# Autodesk Inventor assembly: Automoblox Car assembly
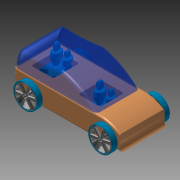
[picture p0: Inventor's stored thumbnail of the model, 180x180]
Saved by Autodesk Inventor 2015 (Build 190159000, 159)
## iProperties
Created: 2014-10-30
Part Number: Automoblox Car assembly
Document SubType Name: Assembly
Designer: cearhart275
Author: cearhart275
## Documents named in this file (14)
- H:\IED II\Automoblox Car assembly.iam
- H:\IED II\Body.ipt
- H:\IED II\Connector Piece.ipt
- H:\IED II\Front.ipt
- H:\IED II\Socket(ellipse Insert).ipt
- H:\IED II\Sockets(Rectangular insert).ipt
- H:\IED II\Tail.ipt
- H:\IED II\Passenger Base.ipt
- H:\IED II\Female Body.ipt
- H:\IED II\Male Figure.ipt
- H:\IED II\Windshield.ipt
- H:\IED II\Axle.ipt
- H:\IED II\Wheel.ipt
- H:\IED II\tire.ipt
## Components (28 placed, 13 different names)
1. Body:1 — Flush:1, Flush:2, Mate:1, Flush:3, Mate:2, Mate:3, Mate:4, Flush:4, Mate:12, Flush:8, Flush:9, Flush:10, Flush:11, Mate:16, Mate:17, Mate:18, Mate:22, Flush:13, Flush:14, Mate:23, Mate:29, Mate:35, Flush:18
2. Socket(ellipse Insert):1 — Flush:1, Flush:2, Mate:1, Flush:3, Mate:2, Mate:5, Mate:6, Mate:19
3. Sockets(Rectangular insert):1 — Mate:3, Mate:4, Flush:4, Mate:7
4. Connector Piece:1 — Mate:5, Mate:6, Mate:19
5. Connector Piece:2 — Mate:7
6. Tail:1 — Mate:8, Mate:9, Mate:10, Flush:5, Flush:6, Flush:7, Mate:11, Mate:12, Flush:8, Flush:9, Flush:10, Flush:11, Mate:13, Mate:14, Mate:15, Mate:26, Mate:32, Mate:36, Insert:3, Insert:4
7. Socket(ellipse Insert):2 — Mate:8, Mate:9, Mate:10, Flush:5, Flush:6, Flush:7, Mate:11
8. Passenger Base:1 — Mate:13, Mate:14, Mate:15, Mate:27, Mate:28, Mate:33, Mate:34, Flush:17
9. Passenger Base:2 — Mate:16, Mate:17, Mate:18, Mate:24, Mate:25, Mate:30, Mate:31, Flush:15, Flush:16
10. Front:1 — Mate:20, Mate:21, Flush:12, Mate:22, Flush:13, Flush:14, Insert:1, Mate:37, Insert:2
11. Sockets(Rectangular insert):2 — Mate:20, Mate:21, Flush:12
12. Male Figure:1 — Mate:23, Mate:24, Mate:25, Flush:16
13. Male Figure:2 — Mate:26, Mate:27, Mate:28
14. Female Body:1 — Mate:29, Mate:30, Mate:31, Flush:15
15. Female Body:2 — Mate:32, Mate:33, Mate:34, Flush:17
16. Windshield:1 — Mate:35, Flush:18, Mate:36
17. Axle:1 — Insert:1, Mate:37, Insert:5
18. Axle:2 — Insert:2, Insert:7
19. Axle:3 — Insert:3, Insert:6
20. Axle:4 — Insert:4, Insert:8
21. Wheel:1 — Mate:38, Flush:19, Insert:5
22. tire:1 — Mate:38, Flush:19
23. tire:2 — Mate:39, Flush:20
24. tire:3 — Mate:41, Flush:22
25. tire:4 — Mate:40, Flush:21
26. Wheel:2 — Mate:40, Flush:21, Insert:8
27. Wheel:3 — Mate:39, Flush:20, Insert:6
28. Wheel:4 — Mate:41, Flush:22, Insert:7
## Relationships (71: Mate 41, Flush 22, Insert 8)
- Flush:1: Body:1 ↔ Socket(ellipse Insert):1
- Flush:2: Body:1 ↔ Socket(ellipse Insert):1
- Mate:1: Body:1 ↔ Socket(ellipse Insert):1
- Flush:3: Body:1 ↔ Socket(ellipse Insert):1
- Mate:2: Body:1 ↔ Socket(ellipse Insert):1
- Mate:3: Body:1 ↔ Sockets(Rectangular insert):1
- Mate:4: Body:1 ↔ Sockets(Rectangular insert):1
- Flush:4: Body:1 ↔ Sockets(Rectangular insert):1
- Mate:5: Socket(ellipse Insert):1 ↔ Connector Piece:1
- Mate:6: Socket(ellipse Insert):1 ↔ Connector Piece:1
- Mate:7: Sockets(Rectangular insert):1 ↔ Connector Piece:2
- Mate:8: Tail:1 ↔ Socket(ellipse Insert):2
- Mate:9: Tail:1 ↔ Socket(ellipse Insert):2
- Mate:10: Tail:1 ↔ Socket(ellipse Insert):2
- Flush:5: Tail:1 ↔ Socket(ellipse Insert):2
- Flush:6: Tail:1 ↔ Socket(ellipse Insert):2
- Flush:7: Tail:1 ↔ Socket(ellipse Insert):2
- Mate:11: Tail:1 ↔ Socket(ellipse Insert):2
- Mate:12: Body:1 ↔ Tail:1
- Flush:8: Body:1 ↔ Tail:1
- Flush:9: Body:1 ↔ Tail:1
- Flush:10: Body:1 ↔ Tail:1
- Flush:11: Body:1 ↔ Tail:1
- Mate:13: Tail:1 ↔ Passenger Base:1
- Mate:14: Tail:1 ↔ Passenger Base:1
- Mate:15: Tail:1 ↔ Passenger Base:1
- Mate:16: Body:1 ↔ Passenger Base:2
- Mate:17: Body:1 ↔ Passenger Base:2
- Mate:18: Body:1 ↔ Passenger Base:2
- Mate:19: Socket(ellipse Insert):1 ↔ Connector Piece:1
- Mate:20: Front:1 ↔ Sockets(Rectangular insert):2
- Mate:21: Front:1 ↔ Sockets(Rectangular insert):2
- Flush:12: Front:1 ↔ Sockets(Rectangular insert):2
- Mate:22: Body:1 ↔ Front:1
- Flush:13: Body:1 ↔ Front:1
- Flush:14: Body:1 ↔ Front:1
- Mate:23: Body:1 ↔ Male Figure:1
- Mate:24: Passenger Base:2 ↔ Male Figure:1
- Mate:25: Passenger Base:2 ↔ Male Figure:1
- Mate:26: Tail:1 ↔ Male Figure:2
- Mate:27: Passenger Base:1 ↔ Male Figure:2
- Mate:28: Passenger Base:1 ↔ Male Figure:2
- Mate:29: Body:1 ↔ Female Body:1
- Mate:30: Passenger Base:2 ↔ Female Body:1
- Mate:31: Passenger Base:2 ↔ Female Body:1
- Flush:15: Passenger Base:2 ↔ Female Body:1
- Flush:16: Passenger Base:2 ↔ Male Figure:1
- Mate:32: Tail:1 ↔ Female Body:2
- Mate:33: Passenger Base:1 ↔ Female Body:2
- Mate:34: Passenger Base:1 ↔ Female Body:2
- Flush:17: Passenger Base:1 ↔ Female Body:2
- Mate:35: Body:1 ↔ Windshield:1
- Flush:18: Body:1 ↔ Windshield:1
- Mate:36: Tail:1 ↔ Windshield:1
- Insert:1: Front:1 ↔ Axle:1
- Mate:37: Front:1 ↔ Axle:1
- Insert:2: Front:1 ↔ Axle:2
- Insert:3: Tail:1 ↔ Axle:3
- Insert:4: Tail:1 ↔ Axle:4
- Mate:38: Wheel:1 ↔ tire:1
- Flush:19: Wheel:1 ↔ tire:1
- Insert:5: Axle:1 ↔ Wheel:1
- Mate:39: tire:2 ↔ Wheel:3
- Flush:20: tire:2 ↔ Wheel:3
- Insert:6: Axle:3 ↔ Wheel:3
- Mate:40: tire:4 ↔ Wheel:2
- Flush:21: tire:4 ↔ Wheel:2
- Mate:41: tire:3 ↔ Wheel:4
- Flush:22: tire:3 ↔ Wheel:4
- Insert:7: Axle:2 ↔ Wheel:4
- Insert:8: Axle:4 ↔ Wheel:2
